# Autodesk Inventor assembly: !gearbox
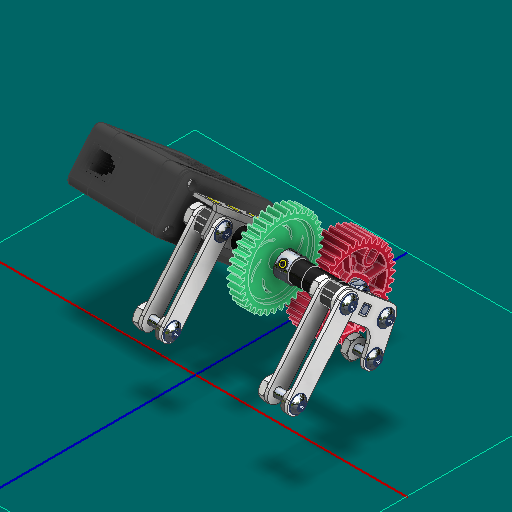
[picture p0: Inventor's stored thumbnail of the model, 512x512]
Saved by Autodesk Inventor 2025 (Build 290162000, 162)
## iProperties
Created: 2024-08-16
Part Number: !gearbox
Document SubType Name: Assembly
Designer: averey
Author: averey
## Documents named in this file (6)
- C:\Users\avere\vex_robotics_high_stakes\hardware\cad\ATLAS\chassis\drive_pod\gearbox\!gearbox.iam
- C:\Users\avere\vex_robotics_high_stakes\hardware\cad\ATLAS\chassis\drive_pod\gearbox\structure.iam
- C:\Users\avere\vex_robotics_high_stakes\hardware\cad\ATLAS\chassis\drive_pod\gearbox\top_shaft.iam
- C:\Users\avere\vex_robotics_high_stakes\hardware\cad\VEX-CAD-Inventor\Electronics\V5 Motor (5.5W).ipt
- C:\Users\avere\vex_robotics_high_stakes\hardware\cad\ATLAS\chassis\drive_pod\gearbox\idler_screw_join.iam
- idler_screw_joint.iam
## Components (4 placed, 4 different names)
1. structure:1 [sub-assembly] — Insert:2, Mate:1, Insert:3, Mate:2, Insert:4
2. top_shaft:1 [sub-assembly] — Angle:1, Insert:4
3. V5 Motor (5.5W):1 — Insert:2, Mate:1, Angle:1
4. idler_screw_joint:1 [sub-assembly] — Insert:3, Mate:2
## Relationships (6: Insert 3, Mate 2, Angle 1)
- Insert:2: structure:1 ↔ V5 Motor (5.5W):1
- Mate:1: structure:1 ↔ V5 Motor (5.5W):1
- Angle:1 (0 deg): top_shaft:1 ↔ V5 Motor (5.5W):1
- Insert:3: structure:1 ↔ idler_screw_joint:1
- Mate:2: structure:1 ↔ idler_screw_joint:1
- Insert:4 (1.27 mm): structure:1 ↔ top_shaft:1
